# Autodesk Inventor assembly: Gear Hub
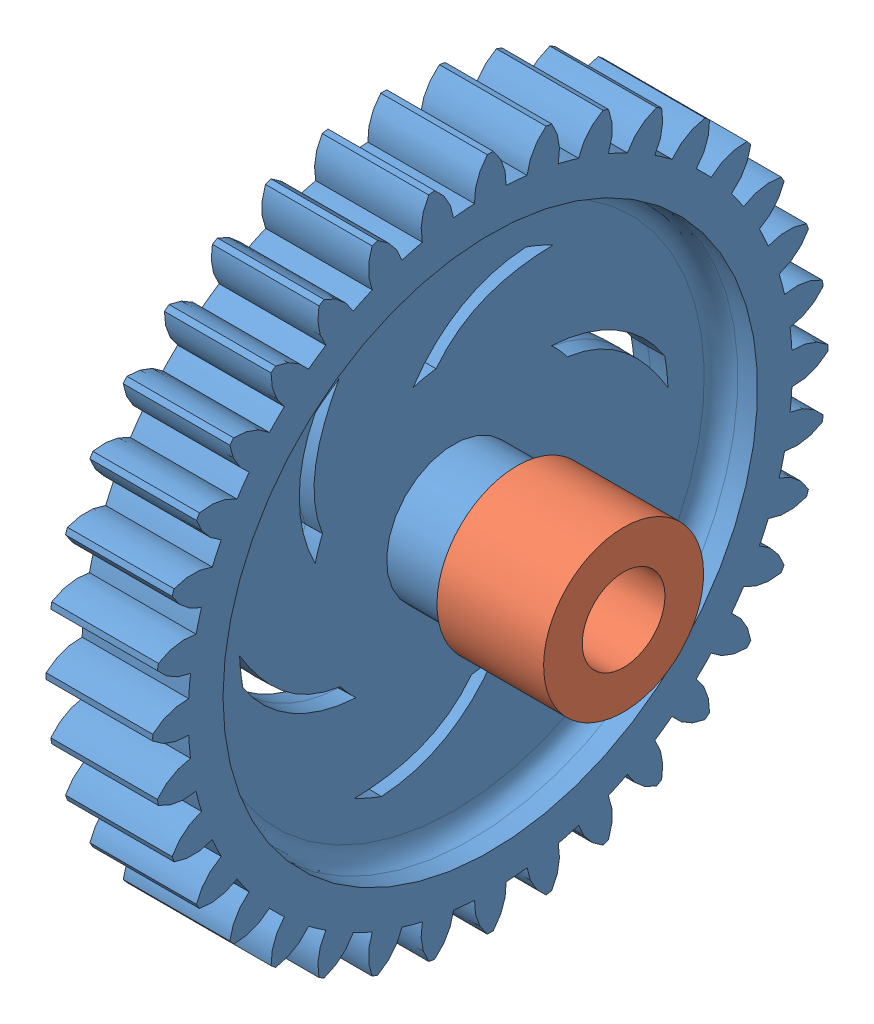
[picture p0: shaded view drawn from the shape stored in the file]
Saved by Autodesk Inventor 2025 (Build 290162000, 162)
## iProperties
Created: 2024-12-18
Part Number: Gear Hub
Document SubType Name: Assembly
Designer: avere
Author: avere
## Documents named in this file (4)
- D:\VEX\High Stakes\CAD\V4\Chassis\Drivebay Left\Gear Hub.iam
- D:\VEX\High Stakes\CAD\ROBOPROS-CAD-Inventor\Motion\Gears\LS 36T Gear.ipt
- D:\VEX\High Stakes\CAD\ROBOPROS-CAD-Inventor\Motion\Spacers\Spacer Nylon .375 OD\NSpacer .375 OD x .250.ipt
- C:\Users\avere\VEX\High Stakes\CAD\ROBOPROS-CAD-Inventor\Motion\Spacers\Spacer Nylon .375 OD.ipt
## Components (2 placed, 2 different names)
1. LS 36T Gear:1
2. NSpacer .375 OD x .250:1
## Relationships (1: Insert 1)
- [Insert]: LS 36T Gear:1 ↔ NSpacer .375 OD x .250:1
